# Autodesk Inventor assembly: Motor_Bar
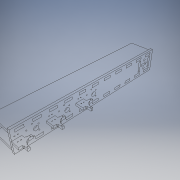
[picture p0: Inventor's stored thumbnail of the model, 180x180]
Saved by Autodesk Inventor 2016 (Build 200138000, 138)
## iProperties
Created: 2016-01-06
Part Number: Motor_Bar
Document SubType Name: Assembly
Designer: m2memari
Author: m2memari
## Documents named in this file (4)
- C:\MoDonGD\Jane\Series_2\Motor_Bar.iam
- C:\MoDonGD\Jane\Series_2\BearingMotorColumn.ipt
- C:\MoDonGD\Jane\Series_2\BearingMotorColumnSupport.ipt
- C:\MoDonGD\Jane\Series_2\BearingStand.ipt
## Components (6 placed, 3 different names)
1. BearingMotorColumn:1 — Mate:1, Mate:2, Mate:3, Mate:4, Mate:5, Mate:6, Mate:7, Mate:8, Mate:9, Mate:10, Mate:11, Mate:12, Mate:13, Mate:14, Mate:15
2. BearingMotorColumnSupport:1 — Mate:1, Mate:2, Mate:3
3. BearingMotorColumnSupport:2 — Mate:4, Mate:5, Mate:6
4. BearingStand:1 — Mate:8, Mate:10, Mate:13
5. BearingStand:2 — Mate:9, Mate:12, Mate:15
6. BearingStand:3 — Mate:7, Mate:11, Mate:14
## Relationships (15: Mate 15)
- Mate:1: BearingMotorColumn:1 ↔ BearingMotorColumnSupport:1
- Mate:2: BearingMotorColumn:1 ↔ BearingMotorColumnSupport:1
- Mate:3: BearingMotorColumn:1 ↔ BearingMotorColumnSupport:1
- Mate:4: BearingMotorColumn:1 ↔ BearingMotorColumnSupport:2
- Mate:5: BearingMotorColumn:1 ↔ BearingMotorColumnSupport:2
- Mate:6: BearingMotorColumn:1 ↔ BearingMotorColumnSupport:2
- Mate:7: BearingMotorColumn:1 ↔ BearingStand:3
- Mate:8: BearingMotorColumn:1 ↔ BearingStand:1
- Mate:9: BearingMotorColumn:1 ↔ BearingStand:2
- Mate:10: BearingMotorColumn:1 ↔ BearingStand:1
- Mate:11: BearingMotorColumn:1 ↔ BearingStand:3
- Mate:12: BearingMotorColumn:1 ↔ BearingStand:2
- Mate:13: BearingMotorColumn:1 ↔ BearingStand:1
- Mate:14: BearingMotorColumn:1 ↔ BearingStand:3
- Mate:15: BearingMotorColumn:1 ↔ BearingStand:2
